# Autodesk Inventor assembly: chassis
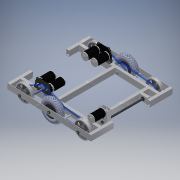
[picture p0: Inventor's stored thumbnail of the model, 180x180]
Saved by Autodesk Inventor 2016 (Build 200138000, 138)
## iProperties
Created: 2016-01-16
Part Number: chassis
Document SubType Name: Assembly
Designer: gus
Mass: 19594.2 g
Surface Area: 37532.9 cm^2
Volume: 8158.93 cm^3
Density: 2.40157 g/cm^3
Author: gus
## Documents named in this file (21)
- C:\Users\Paris\Downloads\Robot-2016-01-20\Robot\chassis\chassis.iam
- C:\Users\Paris\Downloads\Robot-2016-01-20\Robot\chassis\1x2x28.ipt
- C:\Users\Paris\Downloads\Robot-2016-01-20\Robot\chassis\1x2x20.ipt
- C:\Users\Paris\Downloads\Robot-2016-01-20\Robot\chassis\1x2x8in.ipt
- C:\Users\Paris\Downloads\Robot-2016-01-20\Robot\chassis\3 in churro.ipt
- C:\Users\Paris\Downloads\Robot-2016-01-20\Robot\chassis\side plate.ipt
- C:\Users\Paris\Downloads\Robot-2016-01-20\Robot\chassis\PneumaticWheel_am-0970-2.iam
- C:\Users\Paris\Downloads\Robot-2016-01-20\Robot\chassis\CIMple Box\CIMple Box.iam
- C:\Users\Paris\Downloads\Robot-2016-01-20\Robot\chassis\am-0736_S35-12DHE.ipt
- C:\Users\Paris\Downloads\Robot-2016-01-20\Robot\chassis\am-940a-6-HiGrip-.iam
- C:\Users\Paris\Downloads\Robot-2016-01-20\Robot\chassis\half-inch hex bolt.ipt
- C:\Users\Paris\Downloads\Robot-2016-01-20\Robot\chassis\half-inch hex nut.ipt
- C:\Users\Paris\Downloads\Robot-2016-01-20\Robot\chassis\wheel arm support.ipt
- C:\Users\Paris\Downloads\Robot-2016-01-20\Robot\chassis\chassis\Design Accelerator\Chain Drive7.iam
- C:\Users\Paris\Downloads\Robot-2016-01-20\Robot\chassis\chassis\Design Accelerator\Chain Drive8.iam
- C:\Users\Paris\Downloads\Robot-2016-01-20\Robot\chassis\chassis\Design Accelerator\Chain Drive9.iam
- C:\Users\Paris\Downloads\Robot-2016-01-20\Robot\chassis\chassis\Design Accelerator\Chain Drive10.iam
- C:\Users\Paris\Downloads\Robot-2016-01-20\Robot\chassis\chassis\Design Accelerator\Chain Drive11.iam
- C:\Users\Paris\Downloads\Robot-2016-01-20\Robot\chassis\chassis\Design Accelerator\Chain Drive12.iam
- C:\Users\Paris\Downloads\Robot-2016-01-20\Robot\roller wheels\toughbox micro\Toughbox+Nano+All+Shafts+v2-2.iam
- C:\Users\Paris\Downloads\Robot-2016-01-20\Robot\roller wheels\hex bearing.ipt
## Components (45 placed, 15 different names)
1. 1x2x28:1 — Mate:1, Mate:2, Flush:1, Flush:2, Mate:4, Flush:4, Flush:6, Flush:12, Flush:13, Mate:19, Rotational:7, Rotational:8, Cylindrical:25, Rotational:18, Rotational:29, Cylindrical:22, Mate:41, Flush:31, Mate:43, Mate:48
2. 1x2x20:1 — Mate:1, Flush:2, Mate:12, Mate:13, Flush:22, Mate:51, Mate:52
3. 1x2x20:2 — Mate:2, Flush:1, Mate:34, Flush:26, Flush:27, Flush:33
4. 1x2x8in:1 — Mate:8, Flush:9, Flush:10, Mate:13, Mate:35
5. 1x2x8in:2 — Mate:4, Flush:4, Flush:6, Mate:9, Flush:8, Flush:11, Mate:12
6. 3 in churro:1 — Mate:10, Flush:13
7. 3 in churro:2 — Mate:11, Flush:12
8. 3 in churro:3 — Flush:23, Mate:36
9. 3 in churro:4 — Flush:24, Mate:37
10. side plate:1 — Mate:8, Flush:9, Flush:10, Mate:21, Flush:17, Rotational:23, Rotational:24, Rotational:25
11. side plate:2 — Mate:9, Flush:8, Flush:11, Mate:10, Mate:11, Mate:22, Flush:16, Rotational:26, Rotational:27, Rotational:28
12. PneumaticWheel_am-0970-2:1 [sub-assembly] — Rotational:20
13. 1x2x8in:3 — Mate:19, Mate:22, Flush:16, Mate:53, Flush:34
14. 1x2x8in:4 — Mate:21, Flush:17, Mate:33, Flush:20, Flush:21, Flush:28, Mate:39
15. am-0736_S35-12DHE:1 — Cylindrical:2, Mate:49
16. am-0736_S35-12DHE:2 — Mate:50, Cylindrical:26
17. am-940a-6-HiGrip-:1 [sub-assembly] — Cylindrical:25, Mate:48
18. am-940a-6-HiGrip-:2 [sub-assembly] — Cylindrical:22, Mate:43
19. am-940a-6-HiGrip-:3 [sub-assembly] — Cylindrical:23, Mate:45
20. am-940a-6-HiGrip-:4 [sub-assembly] — Cylindrical:24, Mate:44
21. half-inch hex bolt:2 — Rotational:12
22. half-inch hex bolt:4 — Rotational:14
23. half-inch hex bolt:5 — Rotational:7
24. half-inch hex bolt:6 — Rotational:8
25. PneumaticWheel_am-0970-2:2 [sub-assembly] — Rotational:29
26. 1x2x28:2 — Mate:33, Flush:20, Mate:34, Flush:21, Mate:35, Flush:22, Flush:23, Flush:24, Mate:36, Mate:37, Rotational:12, Rotational:14, Cylindrical:24, Rotational:17, Rotational:20, Cylindrical:23, Mate:42, Flush:32, Mate:44, Mate:45
27. half-inch hex bolt:7 — Rotational:17
28. half-inch hex bolt:8 — Rotational:18
29. half-inch hex nut:1 — Rotational:23
30. half-inch hex nut:2 — Rotational:27
31. half-inch hex nut:3 — Rotational:25
32. half-inch hex nut:4 — Rotational:26
33. half-inch hex nut:5 — Rotational:28
34. half-inch hex nut:6 — Rotational:24
35. wheel arm support:1 — Flush:26, Flush:27, Flush:28, Mate:39, Rotational:30
36. CIMple Box:1 [sub-assembly] — Mate:41, Flush:31, Mate:50, Cylindrical:26, Mate:51
37. CIMple Box:2 [sub-assembly] — Mate:42, Flush:32, Cylindrical:2, Mate:49, Mate:52
38. Chain Drive:1 [sub-assembly]
39. Chain Drive:2 [sub-assembly]
40. Chain Drive:3 [sub-assembly]
41. Chain Drive:4 [sub-assembly]
42. Chain Drive:5 [sub-assembly]
43. Chain Drive:6 [sub-assembly]
44. Toughbox+Nano+All+Shafts+v2-2:1 [sub-assembly] — Flush:33, Mate:53, Flush:34, Mate:54
45. hex bearing:1 — Rotational:30, Mate:54
## Relationships (75: Mate 30, Flush 24, RevoluteJoint 15, CylindricalJoint 6)
- Mate:1: 1x2x28:1 ↔ 1x2x20:1
- Mate:2: 1x2x28:1 ↔ 1x2x20:2
- Flush:1: 1x2x28:1 ↔ 1x2x20:2
- Flush:2: 1x2x28:1 ↔ 1x2x20:1
- Mate:4: 1x2x28:1 ↔ 1x2x8in:2
- Flush:4: 1x2x28:1 ↔ 1x2x8in:2
- Flush:6 (88.9 mm): 1x2x28:1 ↔ 1x2x8in:2
- Mate:8: 1x2x8in:1 ↔ side plate:1
- Mate:9: 1x2x8in:2 ↔ side plate:2
- Flush:8: 1x2x8in:2 ↔ side plate:2
- Flush:9: 1x2x8in:1 ↔ side plate:1
- Flush:10: 1x2x8in:1 ↔ side plate:1
- Flush:11: 1x2x8in:2 ↔ side plate:2
- Mate:10: 3 in churro:1 ↔ side plate:2
- Mate:11: 3 in churro:2 ↔ side plate:2
- Mate:12 (304.8 mm): 1x2x20:1 ↔ 1x2x8in:2
- Mate:13 (304.8 mm): 1x2x20:1 ↔ 1x2x8in:1
- Flush:12 (22.225 mm): 1x2x28:1 ↔ 3 in churro:2
- Flush:13 (22.225 mm): 1x2x28:1 ↔ 3 in churro:1
- Mate:19: 1x2x28:1 ↔ 1x2x8in:3
- Mate:21: side plate:1 ↔ 1x2x8in:4
- Mate:22: side plate:2 ↔ 1x2x8in:3
- Flush:16: side plate:2 ↔ 1x2x8in:3
- Flush:17: side plate:1 ↔ 1x2x8in:4
- Rotational:7 [RevoluteJoint]: 1x2x28:1 ↔ half-inch hex bolt:5
- Rotational:8 [RevoluteJoint]: 1x2x28:1 ↔ half-inch hex bolt:6
- Mate:33: 1x2x8in:4 ↔ 1x2x28:2
- Flush:20: 1x2x8in:4 ↔ 1x2x28:2
- Mate:34: 1x2x20:2 ↔ 1x2x28:2
- Flush:21 (88.9 mm): 1x2x8in:4 ↔ 1x2x28:2
- Mate:35: 1x2x8in:1 ↔ 1x2x28:2
- Flush:22: 1x2x20:1 ↔ 1x2x28:2
- Flush:23 (22.225 mm): 3 in churro:3 ↔ 1x2x28:2
- Flush:24 (22.225 mm): 3 in churro:4 ↔ 1x2x28:2
- Mate:36: 3 in churro:3 ↔ 1x2x28:2
- Mate:37: 3 in churro:4 ↔ 1x2x28:2
- Rotational:12 [RevoluteJoint]: half-inch hex bolt:2 ↔ 1x2x28:2
- Rotational:14 [RevoluteJoint]: half-inch hex bolt:4 ↔ 1x2x28:2
- Cylindrical:22: 1x2x28:1 ↔ am-940a-6-HiGrip-:2
- Cylindrical:24: am-940a-6-HiGrip-:4 ↔ 1x2x28:2
- Cylindrical:23: am-940a-6-HiGrip-:3 ↔ 1x2x28:2
- Cylindrical:25: 1x2x28:1 ↔ am-940a-6-HiGrip-:1
- Rotational:17 [RevoluteJoint]: 1x2x28:2 ↔ half-inch hex bolt:7
- Rotational:18 [RevoluteJoint]: 1x2x28:1 ↔ half-inch hex bolt:8
- Rotational:20 [RevoluteJoint]: PneumaticWheel_am-0970-2:1 ↔ 1x2x28:2
- Rotational:29 [RevoluteJoint]: 1x2x28:1 ↔ PneumaticWheel_am-0970-2:2
- Rotational:23 [RevoluteJoint]: side plate:1 ↔ half-inch hex nut:1
- Rotational:24 [RevoluteJoint]: side plate:1 ↔ half-inch hex nut:6
- Rotational:25 [RevoluteJoint]: side plate:1 ↔ half-inch hex nut:3
- Rotational:26 [RevoluteJoint]: side plate:2 ↔ half-inch hex nut:4
- Rotational:27 [RevoluteJoint]: side plate:2 ↔ half-inch hex nut:2
- Rotational:28 [RevoluteJoint]: side plate:2 ↔ half-inch hex nut:5
- Flush:26: 1x2x20:2 ↔ wheel arm support:1
- Flush:27 (-10.0076 mm): 1x2x20:2 ↔ wheel arm support:1
- Flush:28: 1x2x8in:4 ↔ wheel arm support:1
- Mate:39: 1x2x8in:4 ↔ wheel arm support:1
- Mate:41: 1x2x28:1 ↔ CIMple Box:1
- Mate:42: 1x2x28:2 ↔ CIMple Box:2
- Flush:31: 1x2x28:1 ↔ CIMple Box:1
- Flush:32: 1x2x28:2 ↔ CIMple Box:2
- Cylindrical:2: am-0736_S35-12DHE:1 ↔ CIMple Box:2
- Mate:43 (19.1262 mm): 1x2x28:1 ↔ am-940a-6-HiGrip-:2
- Mate:44 (19.1262 mm): am-940a-6-HiGrip-:4 ↔ 1x2x28:2
- Mate:45 (19.1262 mm): am-940a-6-HiGrip-:3 ↔ 1x2x28:2
- Mate:48 (19.1262 mm): 1x2x28:1 ↔ am-940a-6-HiGrip-:1
- Mate:49: am-0736_S35-12DHE:1 ↔ CIMple Box:2
- Mate:50: am-0736_S35-12DHE:2 ↔ CIMple Box:1
- Cylindrical:26: am-0736_S35-12DHE:2 ↔ CIMple Box:1
- Mate:51 (25.4 mm): 1x2x20:1 ↔ CIMple Box:1
- Mate:52 (25.4 mm): 1x2x20:1 ↔ CIMple Box:2
- Flush:33: 1x2x20:2 ↔ Toughbox+Nano+All+Shafts+v2-2:1
- Mate:53: 1x2x8in:3 ↔ Toughbox+Nano+All+Shafts+v2-2:1
- Flush:34: 1x2x8in:3 ↔ Toughbox+Nano+All+Shafts+v2-2:1
- Rotational:30 [RevoluteJoint]: wheel arm support:1 ↔ hex bearing:1
- Mate:54: Toughbox+Nano+All+Shafts+v2-2:1 ↔ hex bearing:1
